# Autodesk Inventor assembly: BottomLaserMountGear
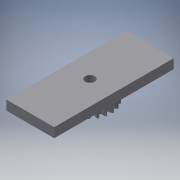
[picture p0: Inventor's stored thumbnail of the model, 180x180]
Saved by Autodesk Inventor 2019 (Build 230136000, 136)
## iProperties
Created: 2019-05-18
Part Number: BottomLaserMountGear
Document SubType Name: Assembly
Designer: Henry
Author: Henry
## Documents named in this file (3)
- D:\Projects\Lidar Scanner\Inventor\FinalMount\BottomLaserMountGear.iam
- D:\Projects\Lidar Scanner\Inventor\FinalMount\LaserMoutBottom.ipt
- D:\Projects\Lidar Scanner\Inventor\SmallGear.ipt
## Components (2 placed, 2 different names)
1. LaserMoutBottom:1 — Cylindrical:1
2. SmallGear:1 — Cylindrical:1
## Relationships (1: CylindricalJoint 1)
- Cylindrical:1: LaserMoutBottom:1 ↔ SmallGear:1
